# Autodesk Inventor assembly: Front_Wheel_Drive
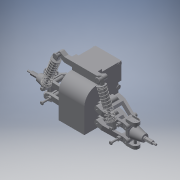
[picture p0: Inventor's stored thumbnail of the model, 180x180]
Saved by Autodesk Inventor 2019 (Build 230136000, 136)
## iProperties
Created: 2019-03-02
Part Number: Front_Wheel_Drive
Document SubType Name: Assembly
Designer: alarr
Author: alarr
## Documents named in this file (14)
- C:\Users\alarr\OneDrive\Documents\Inventor\Mr.Green\Front_Wheel_Drive\Front_Wheel_Drive.iam
- C:\Users\alarr\OneDrive\Documents\Inventor\Mr.Green\Front_Wheel_Drive\Front_Diff.ipt
- C:\Users\alarr\OneDrive\Documents\Inventor\Mr.Green\Front_Wheel_Drive\A_Arm.ipt
- C:\Users\alarr\OneDrive\Documents\Inventor\Mr.Green\Front_Wheel_Drive\A_Arm_MIR.ipt
- C:\Users\alarr\OneDrive\Documents\Inventor\Mr.Green\Shock_Absorber\Shock_Absorber.iam
- C:\Users\alarr\OneDrive\Documents\Inventor\Mr.Green\Front_Wheel_Drive\Steering_Arm.ipt
- C:\Users\alarr\OneDrive\Documents\Inventor\Mr.Green\Front_Wheel_Drive\Arm_Wheel_Attachment.ipt
- C:\Users\alarr\OneDrive\Documents\Inventor\Mr.Green\Front_Wheel_Drive\Front_Wheel_Attachment.ipt
- C:\Users\alarr\OneDrive\Documents\Inventor\Mr.Green\Front_Wheel_Drive\A_Arm_MIR2.ipt
- C:\Users\alarr\OneDrive\Documents\Inventor\Mr.Green\Front_Wheel_Drive\A_Arm_MIR_MIR1.ipt
- C:\Users\alarr\OneDrive\Documents\Inventor\Mr.Green\Shock_Absorber\Shock_Absorber_MIR.iam
- C:\Users\alarr\OneDrive\Documents\Inventor\Mr.Green\Front_Wheel_Drive\Steering_Arm_MIR.ipt
- C:\Users\alarr\OneDrive\Documents\Inventor\Mr.Green\Front_Wheel_Drive\Arm_Wheel_Attachment_MIR.ipt
- C:\Users\alarr\OneDrive\Documents\Inventor\Mr.Green\Front_Wheel_Drive\Front_Wheel_Attachment_MIR.ipt
## Components (13 placed, 13 different names)
1. Front_Diff:1 — Mate:1, Angle:1, Mate:2, Mate:3, Mate:4, Mate:5, Mate:10, Mate:11, Mate:26, Mate:27, Mate:28, Mate:29, Mate:30
2. A_Arm:1 — Mate:2, Mate:3, Mate:12, Mate:14, Mate:17
3. A_Arm_MIR:1 — Mate:4, Mate:5, Mate:13
4. Shock_Absorber:1 [sub-assembly] — Mate:10, Mate:11, Mate:17
5. Steering_Arm:1 — Mate:12, Mate:13, Mate:14, Mate:16, Flush:3
6. Arm_Wheel_Attachment:1 — Flush:1, Flush:2, Mate:15, Mate:16, Flush:3
7. Front_Wheel_Attachment:1 — Flush:2, Mate:15
8. A_Arm_MIR2:1 — Mate:18, Mate:19, Mate:21, Mate:26
9. A_Arm_MIR_MIR1:1 — Mate:20, Mate:27, Mate:28
10. Shock_Absorber_MIR:1 [sub-assembly] — Mate:18, Mate:29, Mate:30
11. Steering_Arm_MIR:1 — Mate:19, Mate:20, Mate:21, Flush:4, Mate:22
12. Arm_Wheel_Attachment_MIR:1 — Flush:4, Mate:22, Mate:23, Mate:24, Mate:25
13. Front_Wheel_Attachment_MIR:1 — Mate:24, Mate:25
## Relationships (31: Mate 26, Flush 4, Angle 1)
- Mate:1: Front_Diff:1
- Angle:1 (0 deg): Front_Diff:1
- Mate:2: Front_Diff:1 ↔ A_Arm:1
- Mate:3: Front_Diff:1 ↔ A_Arm:1
- Mate:4: Front_Diff:1 ↔ A_Arm_MIR:1
- Mate:5: Front_Diff:1 ↔ A_Arm_MIR:1
- Mate:10: Front_Diff:1 ↔ Shock_Absorber:1
- Mate:11: Front_Diff:1 ↔ Shock_Absorber:1
- Mate:12: A_Arm:1 ↔ Steering_Arm:1
- Mate:13: A_Arm_MIR:1 ↔ Steering_Arm:1
- Mate:14: A_Arm:1 ↔ Steering_Arm:1
- Flush:1: Arm_Wheel_Attachment:1
- Flush:2: Arm_Wheel_Attachment:1 ↔ Front_Wheel_Attachment:1
- Mate:15: Arm_Wheel_Attachment:1 ↔ Front_Wheel_Attachment:1
- Mate:16: Steering_Arm:1 ↔ Arm_Wheel_Attachment:1
- Flush:3: Steering_Arm:1 ↔ Arm_Wheel_Attachment:1
- Mate:17: A_Arm:1 ↔ Shock_Absorber:1
- Mate:18: A_Arm_MIR2:1 ↔ Shock_Absorber_MIR:1
- Mate:19: A_Arm_MIR2:1 ↔ Steering_Arm_MIR:1
- Mate:20: A_Arm_MIR_MIR1:1 ↔ Steering_Arm_MIR:1
- Mate:21: A_Arm_MIR2:1 ↔ Steering_Arm_MIR:1
- Flush:4: Steering_Arm_MIR:1 ↔ Arm_Wheel_Attachment_MIR:1
- Mate:22: Steering_Arm_MIR:1 ↔ Arm_Wheel_Attachment_MIR:1
- Mate:23: Arm_Wheel_Attachment_MIR:1
- Mate:24: Arm_Wheel_Attachment_MIR:1 ↔ Front_Wheel_Attachment_MIR:1
- Mate:25: Arm_Wheel_Attachment_MIR:1 ↔ Front_Wheel_Attachment_MIR:1
- Mate:26: Front_Diff:1 ↔ A_Arm_MIR2:1
- Mate:27: Front_Diff:1 ↔ A_Arm_MIR_MIR1:1
- Mate:28: Front_Diff:1 ↔ A_Arm_MIR_MIR1:1
- Mate:29: Front_Diff:1 ↔ Shock_Absorber_MIR:1
- Mate:30: Front_Diff:1 ↔ Shock_Absorber_MIR:1
